# Autodesk Inventor assembly: Part3
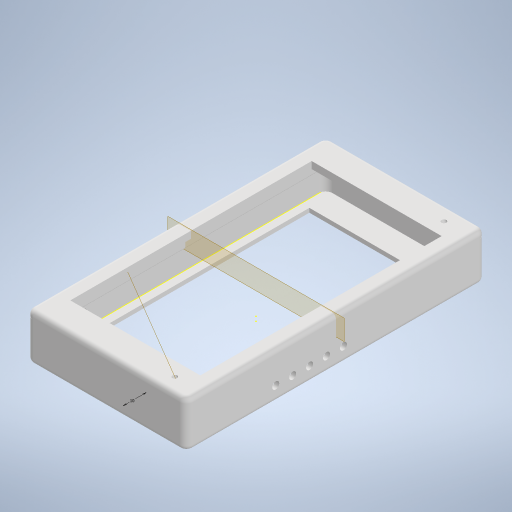
[picture p0: Inventor's stored thumbnail of the model, 512x512]
Saved by Autodesk Inventor 2023 (Build 270158000, 158)
## iProperties
Created: 2022-05-07
Part Number: Part3
Document SubType Name: Assembly
Designer: filip
Author: filip
## Documents named in this file (3)
- C:\Users\filip\Documents\Part3.iam
- C:\Users\filip\Documents\lid.ipt
- C:\Users\filip\Documents\Part3.ipt
## Components (2 placed, 2 different names)
1. lid:1 — Mate:1, Mate:2, Mate:3
2. Part3:1 — Mate:1, Mate:2
## Relationships (3: Mate 3)
- Mate:1: lid:1 ↔ Part3:1
- Mate:2: lid:1 ↔ Part3:1
- Mate:3: lid:1
